# Autodesk Inventor assembly: Left Structure
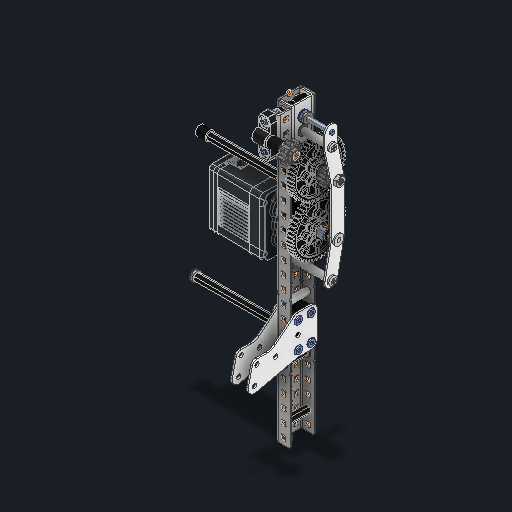
[picture p0: Inventor's stored thumbnail of the model, 512x512]
Saved by Autodesk Inventor 2025.1 (Build 291241000, 241)
## iProperties
Created: 2024-10-20
Part Number: Left Structure
Document SubType Name: Assembly
Designer: Averey Ku
Author: Averey Ku
## Documents named in this file (43)
- C:\Users\avere\VEX\High Stakes\CAD\V3\Tower\Left Structure.iam
- C:\Users\avere\VEX\High Stakes\CAD\ROBOPROS-CAD-Inventor\Structure\C Channel\Aluminum 1x2x1\Alu C 1x2x1x23.ipt
- C:\Users\avere\VEX\High Stakes\CAD\ROBOPROS-CAD-Inventor\Structure\Standoff\Standoff .75.ipt
- C:\Users\avere\VEX\High Stakes\CAD\ROBOPROS-CAD-Inventor\Motion\Spacers\Washer Steel\SWasher .375 OD x .062500.ipt
- C:\Users\avere\VEX\High Stakes\CAD\ROBOPROS-CAD-Inventor\Structure\Standoff\Standoff .875.ipt
- C:\Users\avere\VEX\High Stakes\CAD\ROBOPROS-CAD-Inventor\Structure\Hardware\Nut Nylon\Nut Nylon - White.ipt
- C:\Users\avere\VEX\High Stakes\CAD\ROBOPROS-CAD-Inventor\Motion\Shaft HS\HS Pillow Bearing Block.ipt
- C:\Users\avere\VEX\High Stakes\CAD\ROBOPROS-CAD-Inventor\Structure\Hardware\Screw Steel - Star\SScrew Star Smooth .290.ipt
- C:\Users\avere\VEX\High Stakes\CAD\ROBOPROS-CAD-Inventor\Structure\Hardware\Screw Shoulder Robosource\SScrew Shoulder Smooth .375 x .12.ipt
- C:\Users\avere\VEX\High Stakes\CAD\ROBOPROS-CAD-Inventor\Motion\Spacers\Spacer Nylon .375 OD\NSpacer .375 OD x .250.ipt
- C:\Users\avere\VEX\High Stakes\CAD\ROBOPROS-CAD-Inventor\Motion\Spacers\Spacer Nylon .375 OD\NSpacer .375 OD x .500.ipt
- C:\Users\avere\VEX\High Stakes\CAD\V3\Tower\Custom Parts\Angle Brace Gusset.ipt
- C:\Users\avere\VEX\High Stakes\CAD\ROBOPROS-CAD-Inventor\Structure\Standoff\Standoff .50.ipt
- C:\Users\avere\VEX\High Stakes\CAD\ROBOPROS-CAD-Inventor\Structure\Hardware\Screw Shoulder Robosource\SScrew Shoulder Smooth .290 x .09.ipt
- C:\Users\avere\VEX\High Stakes\CAD\ROBOPROS-CAD-Inventor\Structure\Hardware\Screw Shoulder Robosource\SScrew Shoulder Smooth .500 x .04.ipt
- C:\Users\avere\VEX\High Stakes\CAD\ROBOPROS-CAD-Inventor\Structure\Standoff\Standoff 3.00.ipt
- C:\Users\avere\VEX\High Stakes\CAD\ROBOPROS-CAD-Inventor\Structure\4-Post Standoff Retainer.ipt
- C:\Users\avere\VEX\High Stakes\CAD\ROBOPROS-CAD-Inventor\Structure\Hardware\Screw Steel - Star\SScrew Star Smooth .875.ipt
- C:\Users\avere\VEX\High Stakes\CAD\ROBOPROS-CAD-Inventor\Motion\Spacers\Spacer Nylon .375 OD\NSpacer .375 OD x .375.ipt
- C:\Users\avere\VEX\High Stakes\CAD\ROBOPROS-CAD-Inventor\Structure\Standoff.ipt
- C:\Users\avere\VEX\High Stakes\CAD\ROBOPROS-CAD-Inventor\Motion\Spacers\Washer Steel.ipt
- C:\Users\avere\VEX\High Stakes\CAD\ROBOPROS-CAD-Inventor\Structure\Hardware\Nut Nylon.ipt
- C:\Users\avere\VEX\High Stakes\CAD\ROBOPROS-CAD-Inventor\Structure\Hardware\Screw Steel - Star.ipt
- C:\Users\avere\VEX\High Stakes\CAD\ROBOPROS-CAD-Inventor\Structure\Hardware\Screw Shoulder Robosource.ipt
- C:\Users\avere\VEX\High Stakes\CAD\ROBOPROS-CAD-Inventor\Motion\Spacers\Spacer Nylon .375 OD.ipt
- C:\Users\avere\VEX\High Stakes\CAD\ROBOPROS-CAD-Inventor\Structure\Gussets\C Channel Coupler.ipt
- C:\Users\avere\VEX\High Stakes\CAD\ROBOPROS-CAD-Inventor\Structure\Angle\Aluminum 1x1\Alu Angle 1x1x3.ipt
- C:\Users\avere\VEX\High Stakes\CAD\ROBOPROS-CAD-Inventor\Motion\Spacers\Spacer Nylon .375 OD\NSpacer .375 OD x .125.ipt
- C:\Users\avere\VEX\High Stakes\CAD\ROBOPROS-CAD-Inventor\Motion\Shaft LS\Bearing Flat Low Profile.ipt
- C:\Users\avere\VEX\High Stakes\CAD\ROBOPROS-CAD-Inventor\Structure\Hardware\Screw Steel - Star\SScrew Star Smooth 1.750.ipt
- C:\Users\avere\VEX\High Stakes\CAD\ROBOPROS-CAD-Inventor\Structure\Nylon Standoff Rounded\Nylon Standoff .875.ipt
- C:\Users\avere\VEX\High Stakes\CAD\ROBOPROS-CAD-Inventor\Structure\Hardware\Screw Nylon - Pan Head\NScrew Pan Head Threaded .250.ipt
- C:\Users\avere\VEX\High Stakes\CAD\V3\Intake\Conveyer Gearbox.iam
- C:\Users\avere\VEX\High Stakes\CAD\ROBOPROS-CAD-Inventor\Structure\Hardware\Screw Steel - Star\SScrew Star Smooth 1.250.ipt
- C:\Users\avere\VEX\High Stakes\CAD\ROBOPROS-CAD-Inventor\Structure\Hardware\Nut Keps.ipt
- C:\Users\avere\VEX\High Stakes\CAD\ROBOPROS-CAD-Inventor\Motion\Spacers\Washer Steel\SWasher .375 OD x .015625.ipt
- C:\Users\avere\VEX\High Stakes\CAD\ROBOPROS-CAD-Inventor\Motion\Spacers\Washer Steel\SWasher .375 OD x .031250.ipt
- C:\Users\avere\VEX\High Stakes\CAD\ROBOPROS-CAD-Inventor\Motion\Sprockets\6P Sprocket\6P 8T Sprocket, No Insert.iam
- C:\Users\avere\VEX\High Stakes\CAD\ROBOPROS-CAD-Inventor\Motion\Sprockets\6P Sprocket.iam
- C:\Users\avere\VEX\High Stakes\CAD\ROBOPROS-CAD-Inventor\Motion\Shaft HS\HS Spacer\HSpacer .5000.ipt
- C:\Users\avere\VEX\High Stakes\CAD\ROBOPROS-CAD-Inventor\Motion\Shaft HS\HS Spacer.ipt
- C:\Users\avere\VEX\High Stakes\CAD\ROBOPROS-CAD-Inventor\Electronics\Motors with Screws\SteelM-StarS.iam
- C:\Users\avere\VEX\High Stakes\CAD\ROBOPROS-CAD-Inventor\Electronics\Motors with Screws.iam
## Components (59 placed, 33 different names)
1. Alu C 1x2x1x23:1 — Insert:5, Mate:6, Insert:34, Insert:41, Insert:42, Insert:47, Insert:48, Insert:49, Insert:50, Insert:52, Insert:62, Mate:14
2. NSpacer .375 OD x .375:8 — Insert:32
3. C Channel Coupler:1 — Insert:33, Mate:7, Insert:34, Insert:53, Insert:54
4. Alu Angle 1x1x3:1 — Insert:35, Mate:8, Insert:40, Mate:9
5. SWasher .375 OD x .062500:2 — Insert:38
6. NSpacer .375 OD x .125:9 — Insert:37, Insert:38
7. NSpacer .375 OD x .125:10 — Insert:36, Insert:39
8. Bearing Flat Low Profile:1 — Insert:36, Insert:37, Insert:40
9. SWasher .375 OD x .062500:3 — Insert:39, Mate:9
10. SScrew Star Smooth 1.750:8 — Insert:41
11. SScrew Star Smooth 1.750:9 — Insert:42
12. Nylon Standoff .875:1 — Insert:48
13. Nylon Standoff .875:2 — Insert:47
14. NScrew Pan Head Threaded .250:1 — Insert:49
15. NScrew Pan Head Threaded .250:2 — Insert:50
16. Conveyer Gearbox:1 [sub-assembly] — Insert:52, Mate:13
17. SScrew Star Smooth 1.250:10 — Insert:53
18. Nut Keps:1 — Insert:54, Insert:55
19. SWasher .375 OD x .062500:4 — Insert:55
20. NSpacer .375 OD x .250:11 — Insert:63
21. Standoff 3.00:5
22. SWasher .375 OD x .015625:5
23. SWasher .375 OD x .031250:6
24. SWasher .375 OD x .062500:7
25. 6P 8T Sprocket, No Insert:1 [sub-assembly] — Mate:12, Mate:13
26. HSpacer .5000:1 — Insert:61
27. SteelM-StarS:1 [sub-assembly] — Insert:62, Mate:14
28. Standoff .875:2
29. Nut Nylon - White:1
30. Standoff .75:1
31. SWasher .375 OD x .062500:1
32. SScrew Star Smooth .290:1
33. SScrew Shoulder Smooth .375 x .12:1
34. HS Pillow Bearing Block:1 — Insert:5, Insert:35, Mate:8, Mate:12, Insert:61
35. Nut Nylon - White:2
36. Nut Nylon - White:3
37. NSpacer .375 OD x .250:1
38. NSpacer .375 OD x .500:2 — Insert:33
39. NSpacer .375 OD x .250:3
40. NSpacer .375 OD x .500:4 — Mate:7
41. Angle Brace Gusset:1 — Insert:30
42. Angle Brace Gusset:2 — Insert:31, Insert:63
43. NSpacer .375 OD x .500:5
44. NSpacer .375 OD x .500:6
45. Standoff .50:3
46. NSpacer .375 OD x .500:7
47. SScrew Shoulder Smooth .375 x .12:2
48. SScrew Shoulder Smooth .290 x .09:3
49. SScrew Shoulder Smooth .500 x .04:4
50. Standoff 3.00:4 — Insert:32
51. 4-Post Standoff Retainer:1
52. Nut Nylon - White:4 — Insert:31
53. SScrew Star Smooth .875:4 — Insert:30
54. Nut Nylon - White:5
55. SScrew Star Smooth .875:5
56. Nut Nylon - White:6
57. SScrew Star Smooth .875:6
58. Nut Nylon - White:7
59. SScrew Star Smooth .875:7
## Component patterns: Gusset Mounting Hardware (4 elements)
## Relationships (61: Insert 50, Mate 11)
- [Insert]: Alu C 1x2x1x23:1 ↔ Standoff .75:1
- [Insert]: Standoff .75:1 ↔ SWasher .375 OD x .062500:1
- [Insert]: Alu C 1x2x1x23:1 ↔ Standoff .875:2
- [Insert]: Alu C 1x2x1x23:1 ↔ Nut Nylon - White:1
- Insert:5 (12.7 mm): Alu C 1x2x1x23:1 ↔ HS Pillow Bearing Block:1
- [Mate]: Alu C 1x2x1x23:1 ↔ HS Pillow Bearing Block:1
- [Insert]: Alu C 1x2x1x23:1 ↔ SScrew Star Smooth .290:1
- [Insert]: Alu C 1x2x1x23:1 ↔ SScrew Shoulder Smooth .375 x .12:1
- [Insert]: HS Pillow Bearing Block:1 ↔ Nut Nylon - White:3
- [Insert]: HS Pillow Bearing Block:1 ↔ Nut Nylon - White:2
- [Insert]: NSpacer .375 OD x .250:1 ↔ NSpacer .375 OD x .500:2
- [Insert]: NSpacer .375 OD x .250:3 ↔ NSpacer .375 OD x .500:4
- [Insert] (12.7 mm): Alu C 1x2x1x23:1 ↔ Angle Brace Gusset:1
- [Mate]: Alu C 1x2x1x23:1 ↔ Angle Brace Gusset:1
- [Insert]: Alu C 1x2x1x23:1 ↔ Angle Brace Gusset:2
- [Mate]: Alu C 1x2x1x23:1 ↔ Angle Brace Gusset:2
- [Insert]: Angle Brace Gusset:1 ↔ NSpacer .375 OD x .500:5
- [Insert]: Angle Brace Gusset:1 ↔ NSpacer .375 OD x .500:6
- [Insert]: Angle Brace Gusset:1 ↔ NSpacer .375 OD x .500:7
- [Insert]: Angle Brace Gusset:1 ↔ Standoff .50:3
- [Insert]: Angle Brace Gusset:2 ↔ SScrew Shoulder Smooth .375 x .12:2
- [Insert]: Angle Brace Gusset:1 ↔ SScrew Shoulder Smooth .290 x .09:3
- [Insert]: Alu C 1x2x1x23:1 ↔ SScrew Shoulder Smooth .500 x .04:4
- [Insert]: Alu C 1x2x1x23:1 ↔ 4-Post Standoff Retainer:1
- [Mate]: Alu C 1x2x1x23:1 ↔ 4-Post Standoff Retainer:1
- [Insert]: Standoff 3.00:4 ↔ 4-Post Standoff Retainer:1
- Mate:6: Alu C 1x2x1x23:1
- Insert:30: Angle Brace Gusset:1 ↔ SScrew Star Smooth .875:4
- Insert:31: Angle Brace Gusset:2 ↔ Nut Nylon - White:4
- Insert:32: NSpacer .375 OD x .375:8 ↔ Standoff 3.00:4
- Insert:33: C Channel Coupler:1 ↔ NSpacer .375 OD x .500:2
- Mate:7: C Channel Coupler:1 ↔ NSpacer .375 OD x .500:4
- Insert:34: Alu C 1x2x1x23:1 ↔ C Channel Coupler:1
- Insert:35: Alu Angle 1x1x3:1 ↔ HS Pillow Bearing Block:1
- Mate:8: Alu Angle 1x1x3:1 ↔ HS Pillow Bearing Block:1
- Insert:36 (1.27 mm): NSpacer .375 OD x .125:10 ↔ Bearing Flat Low Profile:1
- Insert:37 (1.27 mm): NSpacer .375 OD x .125:9 ↔ Bearing Flat Low Profile:1
- Insert:38: SWasher .375 OD x .062500:2 ↔ NSpacer .375 OD x .125:9
- Insert:39: NSpacer .375 OD x .125:10 ↔ SWasher .375 OD x .062500:3
- Insert:40: Alu Angle 1x1x3:1 ↔ Bearing Flat Low Profile:1
- Mate:9: Alu Angle 1x1x3:1 ↔ SWasher .375 OD x .062500:3
- Insert:41: Alu C 1x2x1x23:1 ↔ SScrew Star Smooth 1.750:8
- Insert:42: Alu C 1x2x1x23:1 ↔ SScrew Star Smooth 1.750:9
- Insert:47: Alu C 1x2x1x23:1 ↔ Nylon Standoff .875:2
- Insert:48: Alu C 1x2x1x23:1 ↔ Nylon Standoff .875:1
- Insert:49: Alu C 1x2x1x23:1 ↔ NScrew Pan Head Threaded .250:1
- Insert:50: Alu C 1x2x1x23:1 ↔ NScrew Pan Head Threaded .250:2
- Insert:52: Alu C 1x2x1x23:1 ↔ Conveyer Gearbox:1
- Insert:53: C Channel Coupler:1 ↔ SScrew Star Smooth 1.250:10
- Insert:54: C Channel Coupler:1 ↔ Nut Keps:1
- Insert:55: Nut Keps:1 ↔ SWasher .375 OD x .062500:4
- [Insert]: NSpacer .375 OD x .250:11 ↔ Standoff 3.00:5
- [Insert]: SWasher .375 OD x .031250:6 ↔ SWasher .375 OD x .062500:7
- [Insert]: SWasher .375 OD x .015625:5 ↔ SWasher .375 OD x .031250:6
- [Insert]: Standoff 3.00:5 ↔ SWasher .375 OD x .062500:7
- Mate:12: 6P 8T Sprocket, No Insert:1 ↔ HS Pillow Bearing Block:1
- Mate:13: Conveyer Gearbox:1 ↔ 6P 8T Sprocket, No Insert:1
- Insert:61: HSpacer .5000:1 ↔ HS Pillow Bearing Block:1
- Insert:62: Alu C 1x2x1x23:1 ↔ SteelM-StarS:1
- Mate:14: Alu C 1x2x1x23:1 ↔ SteelM-StarS:1
- Insert:63: NSpacer .375 OD x .250:11 ↔ Angle Brace Gusset:2
## Named parameters: d67_d65 = 0 mm, d112_d77 = 0 mm, d113_d78 = 0 mm, d114_d79 = 0 mm, d115_d80 = 0 mm
